# Autodesk Inventor assembly: 2024_Ensamble_AX12
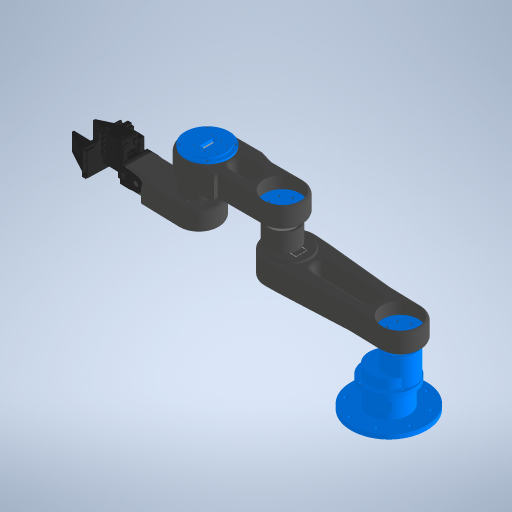
[picture p0: Inventor's stored thumbnail of the model, 512x512]
Saved by Autodesk Inventor 2024 (Build 280153000, 153)
## iProperties
Created: 2022-06-07
Part Number: 2024_Ensamble_AX12
Document SubType Name: Assembly
Designer: Alcatraz
Author: Alcatraz
## Documents named in this file (5)
- C:\Users\Alcatraz\Desktop\TESIS-actual\Lista_Piezas_MovPlano_21Junio\Lista_Piezas\2024_Ensamble_AX12.iam
- C:\Users\Alcatraz\Desktop\TESIS-actual\Lista_Piezas_MovPlano_21Junio\Lista_Piezas\Eslabon_1.iam
- C:\Users\Alcatraz\Desktop\TESIS-actual\Lista_Piezas_MovPlano_21Junio\Lista_Piezas\Eslabon_2.iam
- C:\Users\Alcatraz\Desktop\TESIS-actual\Lista_Piezas_MovPlano_21Junio\Lista_Piezas\Eslabon_3.iam
- C:\Users\Alcatraz\Desktop\TESIS-actual\Lista_Piezas_MovPlano_21Junio\Lista_Piezas\Base-AX12\Base_AX12.iam
## Components (4 placed, 4 different names)
1. Eslabon_1:1 [sub-assembly] — De rotación:1, De rotación:2
2. Eslabon_2:1 [sub-assembly] — De rotación:2, De rotación:3
3. Eslabon_3:1 [sub-assembly] — De rotación:3
4. Base_AX12:1 [sub-assembly] — De rotación:1
## Relationships (3: RevoluteJoint 3)
- De rotación:1 [RevoluteJoint]: Eslabon_1:1 ↔ Base_AX12:1
- De rotación:2 [RevoluteJoint]: Eslabon_1:1 ↔ Eslabon_2:1
- De rotación:3 [RevoluteJoint]: Eslabon_2:1 ↔ Eslabon_3:1
